# Autodesk Inventor assembly: teach_zlozenie_09012023
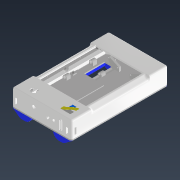
[picture p0: Inventor's stored thumbnail of the model, 180x180]
Saved by Autodesk Inventor 2022 (Build 260153000, 153)
## iProperties
Created: 2023-01-09
Part Number: teach_zlozenie_09012023
Document SubType Name: Assembly
Designer: Simtech
Author: Simtech
## Documents named in this file (17)
- Y:\projekty\!!Simtech - projekty wewnętrzne\!Projekt Mixed Reality\01 Robot Cell (ŚCP)\01 Projekt\08 Pendant\Model CAD\2023 01 09\20230109_0743\teach_zlozenie_09012023.iam
- Y:\projekty\!!Simtech - projekty wewnętrzne\!Projekt Mixed Reality\01 Robot Cell (ŚCP)\01 Projekt\08 Pendant\Model CAD\2023 01 09\20230109_0743\obudowa_przod_tracker_V6.iam
- Y:\projekty\!!Simtech - projekty wewnętrzne\!Projekt Mixed Reality\01 Robot Cell (ŚCP)\01 Projekt\08 Pendant\Model CAD\2023 01 09\20230109_0743\pokrywa_V6.ipt v3.ipt
- Y:\projekty\!!Simtech - projekty wewnętrzne\!Projekt Mixed Reality\01 Robot Cell (ŚCP)\01 Projekt\08 Pendant\Model CAD\2023 01 09\20230109_0743\Uchwyt deadman v3.ipt
- Y:\projekty\!!Simtech - projekty wewnętrzne\!Projekt Mixed Reality\01 Robot Cell (ŚCP)\01 Projekt\08 Pendant\Model CAD\2023 01 09\20230109_0743\uchwyt_usb v1.ipt
- Y:\projekty\!!Simtech - projekty wewnętrzne\!Projekt Mixed Reality\01 Robot Cell (ŚCP)\01 Projekt\08 Pendant\Model CAD\2023 01 09\20230109_0743\belka v1.ipt
- Y:\projekty\!!Simtech - projekty wewnętrzne\!Projekt Mixed Reality\01 Robot Cell (ŚCP)\01 Projekt\08 Pendant\Model CAD\2023 01 09\20230109_0743\DIN 912 - M3 x 0,5 x 30 x 18_x35.ipt
- C:\Users\Simtech\Documents\Inventor\Content Center Files\R2022\pl-PL\DIN 912\DIN 912 - M3 x 0,5 x 20 x 18,75.ipt
- C:\Users\Simtech\Documents\Inventor\Content Center Files\R2022\pl-PL\DIN 985\DIN 985 - M3.ipt
- C:\Users\Simtech\Documents\Inventor\Content Center Files\R2022\pl-PL\DIN 912\DIN 912 - M3 x 0,5 x 10 x 8,75.ipt
- C:\Users\Simtech\Documents\Inventor\Content Center Files\R2022\pl-PL\ISO 10642(1)\ISO 10642 - M3 x  10.ipt
- C:\Users\Simtech\Documents\Inventor\Content Center Files\R2022\pl-PL\DIN 912\DIN 912 - M3 x 0,5 x 8 x 6,75.ipt
- C:\Users\Simtech\Documents\Inventor\Content Center Files\R2022\pl-PL\DIN 128\DIN 128 - A3.ipt
- C:\Users\Simtech\Documents\Inventor\Content Center Files\R2022\pl-PL\DIN 125-1  A\DIN 125 - A 3,2.ipt
- C:\Users\Simtech\Documents\Inventor\Content Center Files\R2022\pl-PL\DIN 934\DIN 934 - M3 x 0,5.ipt
- C:\Users\Simtech\Documents\Inventor\Content Center Files\R2022\pl-PL\DIN 912\DIN 912 - M3 x 0,5 x 16 x 14,75.ipt
- Y:\projekty\!!Simtech - projekty wewnętrzne\!Projekt Mixed Reality\01 Robot Cell (ŚCP)\01 Projekt\08 Pendant\Model CAD\2023 01 09\20230109_0743\Uchwyt deadman v3_prawy.ipt
## Components (40 placed, 16 different names)
1. obudowa_przod_tracker_V6:1 [sub-assembly] — Zestawiające:1, Zestawiające:2, Zestawiające:3, Wstawiające:15, Kątowe:4, Zestawiające:6, Zestawiające:7, Zestawiające:8, Zestawiające:14, Zestawiające:16, Zestawiające:20, Zestawiające:21, Zestawiające:22
2. pokrywa_V6.ipt v3:1 — Zestawiające:1, Zestawiające:2, Zestawiające:3, Wstawiające:2, Zestawiające:5, Wstawiające:5, Wstawiające:6, Wstawiające:10, Kątowe:1, Wstawiające:12, Kątowe:2, Wstawiające:14, Kątowe:3, Wstawiające:28, Zestawiające:28, Zestawiające:29, Równoległe:6, Wstawiające:32, Kątowe:7
3. uchwyt_usb v1:1 — Wstawiające:15, Kątowe:4, Zestawiające:12, Wstawiające:21
4. Uchwyt deadman v3:2 — Wstawiające:2, Zestawiające:5, Wstawiające:9, Wstawiające:11, Wstawiające:13
5. DIN 912 - zastąpiona przez DIN EN ISO 4762 M3 x 30:1 — Wstawiające:5
6. belka v1:1 — Zestawiające:6, Zestawiające:7, Zestawiające:8, Zestawiające:9, Równoległe:1, Zestawiające:10, Zestawiające:11, Wstawiające:22, Kątowe:5, Wstawiające:23, Kątowe:6
7. DIN 912 - zastąpiona przez DIN EN ISO 4762 M3 x 30:3 — Wstawiające:6
8. DIN 912 - zastąpiona przez DIN EN ISO 4762 M3 x 20:1 — Wstawiające:9
9. DIN 985 - zastąpiona przez DIN EN ISO 10511 M3:1 — Wstawiające:10, Kątowe:1
10. DIN 912 - zastąpiona przez DIN EN ISO 4762 M3 x 20:3 — Wstawiające:11
11. DIN 985 - zastąpiona przez DIN EN ISO 10511 M3:3 — Wstawiające:12, Kątowe:2
12. DIN 912 - zastąpiona przez DIN EN ISO 4762 M3 x 10:1 — Wstawiające:13
13. DIN 985 - zastąpiona przez DIN EN ISO 10511 M3:4 — Wstawiające:14, Kątowe:3
14. ISO 10642 M3x10:1 — Zestawiające:9, Równoległe:1, Równoległe:2, Równoległe:3
15. ISO 10642 M3x10:2 — Zestawiające:10, Równoległe:2
16. ISO 10642 M3x10:3 — Zestawiające:11, Równoległe:3
17. DIN 912 - zastąpiona przez DIN EN ISO 4762 M3 x 8:1 — Zestawiające:12, Wstawiające:20
18. DIN 125-1 A A 3,2:2 — Wstawiające:21
19. DIN 128 A3:2 — Wstawiające:20
20. DIN 934 - zastąpiona przez DIN EN 24032/28673/28674 M3:1 — Wstawiające:22, Kątowe:5, Zestawiające:13
21. DIN 934 - zastąpiona przez DIN EN 24032/28673/28674 M3:2 — Wstawiające:23, Kątowe:6, Zestawiające:15
22. DIN 912 - zastąpiona przez DIN EN ISO 4762 M3 x 16:1 — Zestawiające:13, Zestawiające:14
23. DIN 912 - zastąpiona przez DIN EN ISO 4762 M3 x 16:2 — Zestawiające:15, Zestawiające:16
24. belka v1:2 — Zestawiające:20, Zestawiające:21, Zestawiające:22
25. Uchwyt deadman v3_prawy:1 — Zestawiające:28, Zestawiające:29, Równoległe:6, Wstawiające:29, Wstawiające:30, Wstawiające:31
26. DIN 912 - zastąpiona przez DIN EN ISO 4762 M3 x 30:4
27. DIN 912 - zastąpiona przez DIN EN ISO 4762 M3 x 30:5
28. DIN 912 - zastąpiona przez DIN EN ISO 4762 M3 x 20:4 — Wstawiające:31
29. DIN 985 - zastąpiona przez DIN EN ISO 10511 M3:5 — Wstawiające:32, Kątowe:7
30. DIN 912 - zastąpiona przez DIN EN ISO 4762 M3 x 20:5 — Wstawiające:29
31. DIN 985 - zastąpiona przez DIN EN ISO 10511 M3:6
32. DIN 912 - zastąpiona przez DIN EN ISO 4762 M3 x 10:2 — Wstawiające:30
33. DIN 985 - zastąpiona przez DIN EN ISO 10511 M3:7 — Wstawiające:28
34. ISO 10642 M3x10:4 — Równoległe:4, Równoległe:5
35. ISO 10642 M3x10:5 — Równoległe:4
36. ISO 10642 M3x10:6 — Równoległe:5
37. DIN 934 - zastąpiona przez DIN EN 24032/28673/28674 M3:3 — Zestawiające:26
38. DIN 934 - zastąpiona przez DIN EN 24032/28673/28674 M3:4 — Zestawiające:27
39. DIN 912 - zastąpiona przez DIN EN ISO 4762 M3 x 16:3 — Zestawiające:26
40. DIN 912 - zastąpiona przez DIN EN ISO 4762 M3 x 16:4 — Zestawiające:27
## Relationships (56: Mate 22, Insert 21, Angle 7, Flush 6)
- Zestawiające:1 [Mate]: obudowa_przod_tracker_V6:1 ↔ pokrywa_V6.ipt v3:1
- Zestawiające:2 [Mate]: obudowa_przod_tracker_V6:1 ↔ pokrywa_V6.ipt v3:1
- Zestawiające:3 [Mate]: obudowa_przod_tracker_V6:1 ↔ pokrywa_V6.ipt v3:1
- Wstawiające:2 [Insert]: pokrywa_V6.ipt v3:1 ↔ Uchwyt deadman v3:2
- Zestawiające:5 [Mate]: pokrywa_V6.ipt v3:1 ↔ Uchwyt deadman v3:2
- Wstawiające:5 [Insert]: pokrywa_V6.ipt v3:1 ↔ DIN 912 - zastąpiona przez DIN EN ISO 4762 M3 x 30:1
- Wstawiające:6 [Insert]: pokrywa_V6.ipt v3:1 ↔ DIN 912 - zastąpiona przez DIN EN ISO 4762 M3 x 30:3
- Wstawiające:9 [Insert]: Uchwyt deadman v3:2 ↔ DIN 912 - zastąpiona przez DIN EN ISO 4762 M3 x 20:1
- Wstawiające:10 [Insert]: pokrywa_V6.ipt v3:1 ↔ DIN 985 - zastąpiona przez DIN EN ISO 10511 M3:1
- Kątowe:1 [Angle] (0 deg): pokrywa_V6.ipt v3:1 ↔ DIN 985 - zastąpiona przez DIN EN ISO 10511 M3:1
- Wstawiające:11 [Insert]: Uchwyt deadman v3:2 ↔ DIN 912 - zastąpiona przez DIN EN ISO 4762 M3 x 20:3
- Wstawiające:12 [Insert]: pokrywa_V6.ipt v3:1 ↔ DIN 985 - zastąpiona przez DIN EN ISO 10511 M3:3
- Kątowe:2 [Angle] (0 deg): pokrywa_V6.ipt v3:1 ↔ DIN 985 - zastąpiona przez DIN EN ISO 10511 M3:3
- Wstawiające:13 [Insert]: Uchwyt deadman v3:2 ↔ DIN 912 - zastąpiona przez DIN EN ISO 4762 M3 x 10:1
- Wstawiające:14 [Insert]: pokrywa_V6.ipt v3:1 ↔ DIN 985 - zastąpiona przez DIN EN ISO 10511 M3:4
- Kątowe:3 [Angle] (0 deg): pokrywa_V6.ipt v3:1 ↔ DIN 985 - zastąpiona przez DIN EN ISO 10511 M3:4
- Wstawiające:15 [Insert]: obudowa_przod_tracker_V6:1 ↔ uchwyt_usb v1:1
- Kątowe:4 [Angle] (0 deg): obudowa_przod_tracker_V6:1 ↔ uchwyt_usb v1:1
- Zestawiające:6 [Mate]: obudowa_przod_tracker_V6:1 ↔ belka v1:1
- Zestawiające:7 [Mate]: obudowa_przod_tracker_V6:1 ↔ belka v1:1
- Zestawiające:8 [Mate]: obudowa_przod_tracker_V6:1 ↔ belka v1:1
- Zestawiające:9 [Mate]: belka v1:1 ↔ ISO 10642 M3x10:1
- Równoległe:1 [Flush] (2.7 mm): belka v1:1 ↔ ISO 10642 M3x10:1
- Zestawiające:10 [Mate]: belka v1:1 ↔ ISO 10642 M3x10:2
- Równoległe:2 [Flush]: ISO 10642 M3x10:1 ↔ ISO 10642 M3x10:2
- Zestawiające:11 [Mate]: belka v1:1 ↔ ISO 10642 M3x10:3
- Równoległe:3 [Flush]: ISO 10642 M3x10:1 ↔ ISO 10642 M3x10:3
- Zestawiające:12 [Mate]: uchwyt_usb v1:1 ↔ DIN 912 - zastąpiona przez DIN EN ISO 4762 M3 x 8:1
- [Insert]: DIN 125-1 A A 3,2:2 ↔ DIN 128 A3:2
- [Insert]: DIN 125-1 A A 3,2:2 ↔ DIN 128 A3:2
- Wstawiające:20 [Insert]: DIN 912 - zastąpiona przez DIN EN ISO 4762 M3 x 8:1 ↔ DIN 128 A3:2
- Wstawiające:21 [Insert]: uchwyt_usb v1:1 ↔ DIN 125-1 A A 3,2:2
- Wstawiające:22 [Insert]: belka v1:1 ↔ DIN 934 - zastąpiona przez DIN EN 24032/28673/28674 M3:1
- Kątowe:5 [Angle] (0 deg): belka v1:1 ↔ DIN 934 - zastąpiona przez DIN EN 24032/28673/28674 M3:1
- Wstawiające:23 [Insert]: belka v1:1 ↔ DIN 934 - zastąpiona przez DIN EN 24032/28673/28674 M3:2
- Kątowe:6 [Angle] (0 deg): belka v1:1 ↔ DIN 934 - zastąpiona przez DIN EN 24032/28673/28674 M3:2
- Zestawiające:13 [Mate]: DIN 934 - zastąpiona przez DIN EN 24032/28673/28674 M3:1 ↔ DIN 912 - zastąpiona przez DIN EN ISO 4762 M3 x 16:1
- Zestawiające:14 [Mate]: obudowa_przod_tracker_V6:1 ↔ DIN 912 - zastąpiona przez DIN EN ISO 4762 M3 x 16:1
- Zestawiające:15 [Mate]: DIN 934 - zastąpiona przez DIN EN 24032/28673/28674 M3:2 ↔ DIN 912 - zastąpiona przez DIN EN ISO 4762 M3 x 16:2
- Zestawiające:16 [Mate]: obudowa_przod_tracker_V6:1 ↔ DIN 912 - zastąpiona przez DIN EN ISO 4762 M3 x 16:2
- Zestawiające:20 [Mate]: obudowa_przod_tracker_V6:1 ↔ belka v1:2
- Zestawiające:21 [Mate]: obudowa_przod_tracker_V6:1 ↔ belka v1:2
- Zestawiające:22 [Mate]: obudowa_przod_tracker_V6:1 ↔ belka v1:2
- Równoległe:4 [Flush]: ISO 10642 M3x10:4 ↔ ISO 10642 M3x10:5
- Równoległe:5 [Flush]: ISO 10642 M3x10:4 ↔ ISO 10642 M3x10:6
- Zestawiające:26 [Mate]: DIN 934 - zastąpiona przez DIN EN 24032/28673/28674 M3:3 ↔ DIN 912 - zastąpiona przez DIN EN ISO 4762 M3 x 16:3
- Zestawiające:27 [Mate]: DIN 934 - zastąpiona przez DIN EN 24032/28673/28674 M3:4 ↔ DIN 912 - zastąpiona przez DIN EN ISO 4762 M3 x 16:4
- Wstawiające:28 [Insert]: pokrywa_V6.ipt v3:1 ↔ DIN 985 - zastąpiona przez DIN EN ISO 10511 M3:7
- Zestawiające:28 [Mate]: pokrywa_V6.ipt v3:1 ↔ Uchwyt deadman v3_prawy:1
- Zestawiające:29 [Mate]: pokrywa_V6.ipt v3:1 ↔ Uchwyt deadman v3_prawy:1
- Równoległe:6 [Flush]: pokrywa_V6.ipt v3:1 ↔ Uchwyt deadman v3_prawy:1
- Wstawiające:29 [Insert]: Uchwyt deadman v3_prawy:1 ↔ DIN 912 - zastąpiona przez DIN EN ISO 4762 M3 x 20:5
- Wstawiające:30 [Insert]: Uchwyt deadman v3_prawy:1 ↔ DIN 912 - zastąpiona przez DIN EN ISO 4762 M3 x 10:2
- Wstawiające:31 [Insert]: Uchwyt deadman v3_prawy:1 ↔ DIN 912 - zastąpiona przez DIN EN ISO 4762 M3 x 20:4
- Wstawiające:32 [Insert]: pokrywa_V6.ipt v3:1 ↔ DIN 985 - zastąpiona przez DIN EN ISO 10511 M3:5
- Kątowe:7 [Angle] (0 deg): pokrywa_V6.ipt v3:1 ↔ DIN 985 - zastąpiona przez DIN EN ISO 10511 M3:5
## Named parameters: d39_d1006_d996_d388_d378_d106_d90_d72_d68_d18 = 0 mm, d40_d1007_d997_d389_d379_d107_d94_d73_d71_d32 = 0 mm
